# Autodesk Inventor assembly: Bellows Assembly
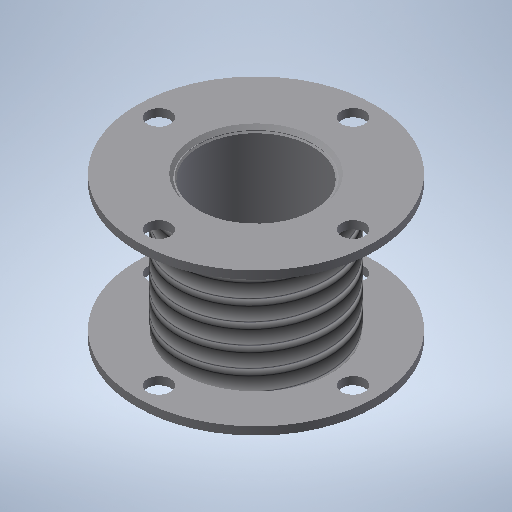
[picture p0: Inventor's stored thumbnail of the model, 512x512]
Saved by Autodesk Inventor 2025 (Build 290162000, 162)
## iProperties
Created: 2021-01-07
Part Number: Bellows Assembly
Document SubType Name: Assembly
Designer: caleb
Author: caleb
## Documents named in this file (3)
- C:\Users\cfang\Desktop\nebraska-silicon-lab\Hardware\ETL\Module Assembly\Picker Tool\Bellows Assembly.iam
- C:\Users\cfang\Desktop\nebraska-silicon-lab\Hardware\ETL\Module Assembly\Picker Tool\FC-13 Bellows.ipt
- C:\Users\cfang\Desktop\nebraska-silicon-lab\Hardware\ETL\Module Assembly\Picker Tool\Flange_1.ipt
## Components (3 placed, 2 different names)
1. FC-13 Bellows:1 — Insert:2, Insert:3
2. Flange_1:1 — Insert:2
3. Flange_1:2 — Insert:3
## Relationships (2: Insert 2)
- Insert:2 (-1.1176 mm): FC-13 Bellows:1 ↔ Flange_1:1
- Insert:3 (-1.118 mm): FC-13 Bellows:1 ↔ Flange_1:2
